# Autodesk Inventor assembly: Z_Gantry_Plate_Spaced
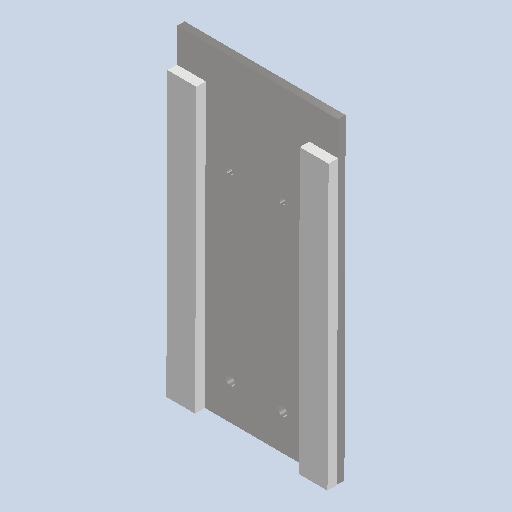
[picture p0: Inventor's stored thumbnail of the model, 512x512]
Saved by Autodesk Inventor 2023 (Build 270158000, 158)
## iProperties
Created: 2022-06-21
Part Number: Z_Gantry_Plate_Spaced
Document SubType Name: Assembly
Designer: plebbb
Author: plebbb
## Documents named in this file (3)
- C:\Users\think\OneDrive\Desktop\CNC_Project\Z_Gantry_Plate_Spaced.iam
- C:\Users\think\OneDrive\Desktop\CNC_Project\Z_Gantry_Plate.ipt
- C:\Users\think\OneDrive\Desktop\CNC_Project\Rail_Spacer_Plate.ipt
## Components (3 placed, 2 different names)
1. Z_Gantry_Plate:1 — Flush:3, Flush:4
2. Rail_Spacer_Plate:1 — Flush:3, Flush:5
3. Rail_Spacer_Plate:2 — Flush:4, Flush:5
## Relationships (5: Flush 3, Mate 2)
- [Mate]: Z_Gantry_Plate:1 ↔ Rail_Spacer_Plate:1
- [Mate]: Z_Gantry_Plate:1 ↔ Rail_Spacer_Plate:2
- Flush:3: Z_Gantry_Plate:1 ↔ Rail_Spacer_Plate:1
- Flush:4: Z_Gantry_Plate:1 ↔ Rail_Spacer_Plate:2
- Flush:5: Rail_Spacer_Plate:1 ↔ Rail_Spacer_Plate:2
